# Autodesk Inventor assembly: Refined Piano Hinge
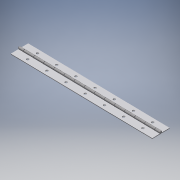
[picture p0: Inventor's stored thumbnail of the model, 180x180]
Saved by Autodesk Inventor 2019 (Build 230136000, 136)
## iProperties
Created: 2019-01-26
Part Number: Refined Piano Hinge
Document SubType Name: Assembly
Designer: josh
Mass: 274.674 g
Surface Area: 1856.56 cm^2
Volume: 274.674 cm^3
Density: 1 g/cm^3
Author: josh
## Documents named in this file (3)
- D:\Synthesis Robots\Epsilon\Chasis\Hinge\Refined Piano Hinge.iam
- D:\Synthesis Robots\Epsilon\Chasis\Hinge\Piano hingehinge - Copy.ipt
- D:\Synthesis Robots\Epsilon\Chasis\Hinge\Piano hingehinge pin - Copy.ipt
## Components (3 placed, 2 different names)
1. Piano hingehinge - Copy:1 — Mate:3, Mate:4
2. Piano hingehinge - Copy:2 — Mate:1, Mate:4, Mate:5
3. Piano hingehinge pin - Copy:1 — Mate:1, Mate:3, Mate:5
## Relationships (4: Mate 4)
- Mate:1: Piano hingehinge - Copy:2 ↔ Piano hingehinge pin - Copy:1
- Mate:3: Piano hingehinge - Copy:1 ↔ Piano hingehinge pin - Copy:1
- Mate:4: Piano hingehinge - Copy:1 ↔ Piano hingehinge - Copy:2
- Mate:5: Piano hingehinge - Copy:2 ↔ Piano hingehinge pin - Copy:1
